# Autodesk Inventor assembly: Assembly1
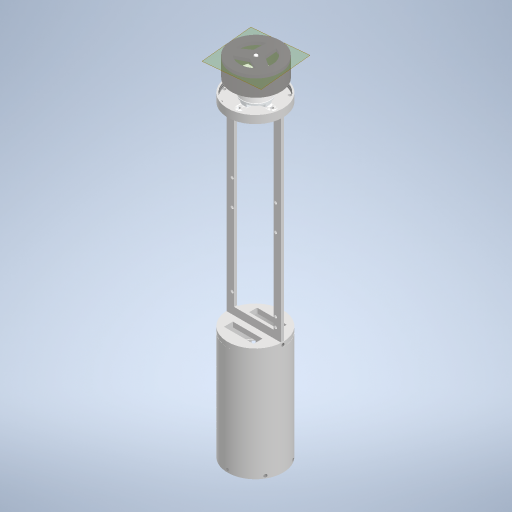
[picture p0: Inventor's stored thumbnail of the model, 512x512]
Saved by Autodesk Inventor 2023 (Build 270158000, 158)
## iProperties
Created: 2022-07-12
Part Number: Assembly1
Document SubType Name: Assembly
Designer: samlo
Author: samlo
## Documents named in this file (5)
- D:\Documents\reaction-wheel\CAD\Assembly1.iam
- D:\Documents\reaction-wheel\CAD\battery holder.ipt
- D:\Documents\reaction-wheel\CAD\case v0.ipt
- D:\Documents\reaction-wheel\CAD\motorMotor_BLDC_2212,6T_2200KV__With_Support.ipt
- D:\Downloads\Reaction_wheel_dr - Copy (3.3) (1).ipt
## Components (4 placed, 4 different names)
1. battery holder:1 — Mate:1
2. case v0:1 — Mate:1, Cylindrical:1
3. motorMotor_BLDC_2212,6T_2200KV__With_Support:1 — Cylindrical:1, Rotational:1
4. Reaction_wheel_dr - Copy (3.3) (1):1 — Rotational:1
## Relationships (3: Mate 1, CylindricalJoint 1, RevoluteJoint 1)
- Mate:1: battery holder:1 ↔ case v0:1
- Cylindrical:1: case v0:1 ↔ motorMotor_BLDC_2212,6T_2200KV__With_Support:1
- Rotational:1 [RevoluteJoint]: motorMotor_BLDC_2212,6T_2200KV__With_Support:1 ↔ Reaction_wheel_dr - Copy (3.3) (1):1
